# Autodesk Inventor assembly: GE-13025
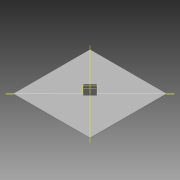
[picture p0: Inventor's stored thumbnail of the model, 180x180]
Saved by Autodesk Inventor 2013 (Build 170138000, 138)
## iProperties
Created: 2013-01-06
Part Number: GE-13025
Document SubType Name: Assembly
Designer: Phillip
Author: Phillip
## Documents named in this file (3)
- E:\Data Folder\FIRST 2013\FIRST KOP\FIRST Arena 2013\Pyramid\GE-13025.iam
- E:\Data Folder\FIRST 2013\FIRST KOP\FIRST Arena 2013\Pyramid\GE-13025-01.ipt
- E:\Data Folder\FIRST 2013\FIRST KOP\FIRST Arena 2013\Pyramid\GE-13025-02.ipt
## Components (2 placed, 2 different names)
1. GE-13025-01:1 — Mate:1, Mate:2, Mate:3, Mate:4, Mate:6, Mate:7, Mate:8
2. GE-13025-02:1 — Mate:1, Mate:5, Mate:9
## Relationships (9: Mate 9)
- Mate:1: GE-13025-01:1 ↔ GE-13025-02:1
- Mate:2: GE-13025-01:1
- Mate:3: GE-13025-01:1
- Mate:4: GE-13025-01:1
- Mate:5: GE-13025-02:1
- Mate:6: GE-13025-01:1
- Mate:7: GE-13025-01:1
- Mate:8: GE-13025-01:1
- Mate:9: GE-13025-02:1
